# Autodesk Inventor assembly: сборка микроконтроллера
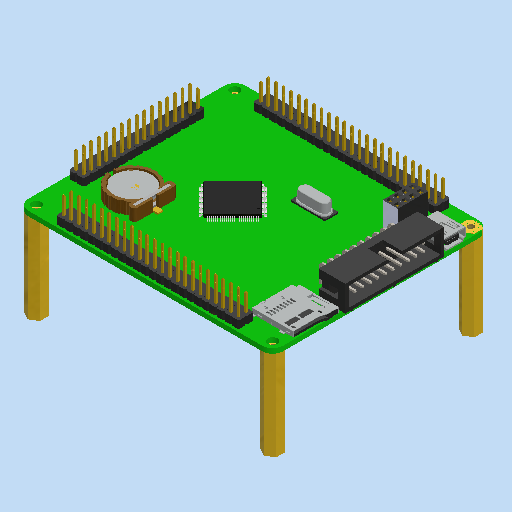
[picture p0: Inventor's stored thumbnail of the model, 512x512]
Saved by Autodesk Inventor 2025 (Build 290162000, 162)
## iProperties
Created: 2025-03-03
Part Number: сборка микроконтроллера
Document SubType Name: Assembly
Designer: volko
Author: volko
## Documents named in this file (3)
- C:\Users\volko\Desktop\диплом\Модели\детали\сборка микроконтроллера.iam
- C:\Users\volko\Desktop\диплом\Модели\детали\втулки крепления электроники.ipt
- C:\Users\volko\Desktop\диплом\Модели\детали\stm32.ipt
## Components (5 placed, 2 different names)
1. втулки крепления электроники:1 — Совмещение:3, Совмещение:6
2. втулки крепления электроники:2 — Совмещение:2, Совмещение:5
3. втулки крепления электроники:3 — Совмещение:7, Совмещение:8
4. втулки крепления электроники:4 — Совмещение:1, Совмещение:4
5. stm32:1 — Совмещение:1, Совмещение:2, Совмещение:3, Совмещение:4, Совмещение:5, Совмещение:6, Совмещение:7, Совмещение:8, Заподлицо:1, Заподлицо:2, Заподлицо:3
## Relationships (11: Mate 8, Flush 3)
- Совмещение:1 [Mate]: втулки крепления электроники:4 ↔ stm32:1
- Совмещение:2 [Mate]: втулки крепления электроники:2 ↔ stm32:1
- Совмещение:3 [Mate]: втулки крепления электроники:1 ↔ stm32:1
- Совмещение:4 [Mate]: втулки крепления электроники:4 ↔ stm32:1
- Совмещение:5 [Mate]: втулки крепления электроники:2 ↔ stm32:1
- Совмещение:6 [Mate]: втулки крепления электроники:1 ↔ stm32:1
- Совмещение:7 [Mate]: втулки крепления электроники:3 ↔ stm32:1
- Совмещение:8 [Mate]: втулки крепления электроники:3 ↔ stm32:1
- Заподлицо:1 [Flush]: stm32:1
- Заподлицо:2 [Flush]: stm32:1
- Заподлицо:3 [Flush]: stm32:1
